# Autodesk Inventor assembly: Assembly1
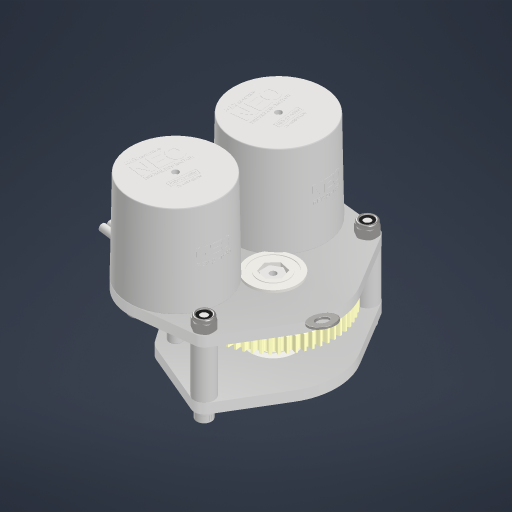
[picture p0: Inventor's stored thumbnail of the model, 512x512]
Saved by Autodesk Inventor 2024.3 (Build 283343000, 343)
## iProperties
Created: 2024-11-01
Part Number: Assembly1
Document SubType Name: Assembly
Designer: kaito
Author: kaito
## Documents named in this file (14)
- C:\Users\kaito\OneDrive\Documents\GitHub\1622-2024-Assignments\Kaito Kubota-Valme\Gearbox 2 v.2\Assembly1.iam
- C:\Users\kaito\OneDrive\Documents\GitHub\1622-2024-Assignments\Kaito Kubota-Valme\Gearbox 2 v.2\Bottom Plate.ipt
- C:\Users\kaito\OneDrive\Documents\GitHub\1622-2024-Assignments\Kaito Kubota-Valme\Gearbox 2 v.2\Part1.ipt
- C:\Users\kaito\OneDrive\Desktop\COTS Library\Motion\Bearings\COTS_WCP-0783_1.125ODHexBearing.ipt
- C:\Users\kaito\OneDrive\Desktop\COTS Library\Motion\Gears\Motor Gears\COTS_217-6334_10T20DPMotorGear.ipt
- C:\Users\kaito\Downloads\REV-21-1650-V1.1\REV-21-1650-V1.1\REV-21-1650-V1.1.ipt
- C:\Users\kaito\OneDrive\Documents\GitHub\1622-2024-Assignments\Kaito Kubota-Valme\Gearbox 2 v.2\Standoff.ipt
- C:\Users\kaito\OneDrive\Documents\GitHub\1622-2024-Assignments\Kaito Kubota-Valme\Gearbox 2 v.2\Hex Shaft.ipt
- C:\Users\kaito\Downloads\WCP-0720 (2)\WCP-0720 (2)\WCP-0720 (2).ipt
- C:\Users\kaito\OneDrive\Desktop\COTS Library\Fasteners\Bolts\Button-Head\10-32\COTS_92949A263_3-8in long Stainless Steel Button Head Screw.ipt
- C:\Users\kaito\OneDrive\Desktop\COTS Library\Fasteners\Washers\COTS_90107A029_316 Stainless Steel Washer.ipt
- C:\Users\kaito\Downloads\91251A550_Black-Oxide Alloy Steel Socket Head Screw\91251A550_Black-Oxide Alloy Steel Socket Head Screw\91251A550_Black-Oxide Alloy Steel Socket Head Screw.ipt
- C:\Users\kaito\OneDrive\Documents\GitHub\1622-2024-Assignments\COTS Library\Fasteners\Nuts\COTS_95615A120_Medium-Strength Steel Nylon-Insert Locknut.ipt
- C:\Users\kaito\OneDrive\Documents\GitHub\1622-2024-Assignments\COTS Library\Fasteners\Washers\COTS_90107A029_316 Stainless Steel Washer.ipt
## Components (28 placed, 12 different names)
1. Bottom Plate:1 — Mate:5, Mate:15, Mate:16, Mate:17, Mate:19, Mate:21, Mate:24, Mate:25, Mate:45, Mate:47, Mate:49
2. Part1:1 — Mate:2, Mate:3, Mate:5, Mate:6, Mate:7, Mate:8, Mate:9, Mate:10, Mate:12, Mate:14, Mate:17, Mate:18, Mate:20, Mate:22, Mate:23, Mate:29, Mate:30, Mate:31, Mate:32, Mate:33, Mate:34, Mate:35, Mate:36, Mate:37, Mate:38, Mate:39, Mate:40, Mate:51, Mate:53, Mate:55
3. COTS_WCP-0783_1.125ODHexBearing:1 — Mate:2, Mate:3, Mate:28
4. COTS_217-6334_10T20DPMotorGear:1 — Mate:13, Mate:14
5. COTS_217-6334_10T20DPMotorGear:2 — Mate:11, Mate:12
6. REV-21-1650-V1.1:1 — Mate:6, Mate:7, Mate:8, Mate:11
7. REV-21-1650-V1.1:2 — Mate:9, Mate:10, Mate:13, Mate:23
8. Standoff:1 — Mate:21, Mate:22, Mate:44
9. Standoff:2 — Mate:15, Mate:16, Mate:18, Mate:48
10. Standoff:3 — Mate:19, Mate:20, Mate:46
11. Hex Shaft:1 — Mate:26, Flush:1, Mate:27, Rotation:1, Mate:42
12. COTS_WCP-0783_1.125ODHexBearing:2 — Mate:24, Mate:25, Mate:26, Flush:1, Mate:41
13. WCP-0720 (2):1 — Mate:27, Mate:28
14. COTS_92949A263_3-8in long Stainless Steel Button Head Screw:1 — Mate:29, Mate:30
15. COTS_92949A263_3-8in long Stainless Steel Button Head Screw:2 — Mate:42, Mate:43
16. COTS_92949A263_3-8in long Stainless Steel Button Head Screw:4 — Mate:31, Mate:32
17. COTS_92949A263_3-8in long Stainless Steel Button Head Screw:5 — Mate:39, Mate:40
18. COTS_92949A263_3-8in long Stainless Steel Button Head Screw:6 — Mate:37, Mate:38
19. COTS_92949A263_3-8in long Stainless Steel Button Head Screw:7 — Mate:35, Mate:36
20. COTS_92949A263_3-8in long Stainless Steel Button Head Screw:8 — Mate:33, Mate:34
21. COTS_90107A029_316 Stainless Steel Washer:1 — Rotation:1, Mate:41, Mate:43
22. 91251A550_Black-Oxide Alloy Steel Socket Head Screw:1 — Mate:44, Mate:45, Mate:54
23. 91251A550_Black-Oxide Alloy Steel Socket Head Screw:2 — Mate:46, Mate:47, Mate:50
24. 91251A550_Black-Oxide Alloy Steel Socket Head Screw:3 — Mate:48, Mate:49, Mate:52
25. COTS_95615A120_Medium-Strength Steel Nylon-Insert Locknut:1 — Mate:50, Mate:51
26. COTS_95615A120_Medium-Strength Steel Nylon-Insert Locknut:2 — Mate:54, Mate:55
27. COTS_95615A120_Medium-Strength Steel Nylon-Insert Locknut:3 — Mate:52, Mate:53
28. COTS_90107A029_316 Stainless Steel Washer:2
## Relationships (55: Mate 53, Flush 1, RelateRotation 1)
- Mate:2: Part1:1 ↔ COTS_WCP-0783_1.125ODHexBearing:1
- Mate:3: Part1:1 ↔ COTS_WCP-0783_1.125ODHexBearing:1
- Mate:5: Bottom Plate:1 ↔ Part1:1
- Mate:6: Part1:1 ↔ REV-21-1650-V1.1:1
- Mate:7: Part1:1 ↔ REV-21-1650-V1.1:1
- Mate:8: Part1:1 ↔ REV-21-1650-V1.1:1
- Mate:9: Part1:1 ↔ REV-21-1650-V1.1:2
- Mate:10: Part1:1 ↔ REV-21-1650-V1.1:2
- Mate:11: COTS_217-6334_10T20DPMotorGear:2 ↔ REV-21-1650-V1.1:1
- Mate:12: Part1:1 ↔ COTS_217-6334_10T20DPMotorGear:2
- Mate:13: COTS_217-6334_10T20DPMotorGear:1 ↔ REV-21-1650-V1.1:2
- Mate:14: Part1:1 ↔ COTS_217-6334_10T20DPMotorGear:1
- Mate:15: Bottom Plate:1 ↔ Standoff:2
- Mate:16: Bottom Plate:1 ↔ Standoff:2
- Mate:17: Bottom Plate:1 ↔ Part1:1
- Mate:18: Part1:1 ↔ Standoff:2
- Mate:19: Bottom Plate:1 ↔ Standoff:3
- Mate:20: Part1:1 ↔ Standoff:3
- Mate:21: Bottom Plate:1 ↔ Standoff:1
- Mate:22: Part1:1 ↔ Standoff:1
- Mate:23: Part1:1 ↔ REV-21-1650-V1.1:2
- Mate:24: Bottom Plate:1 ↔ COTS_WCP-0783_1.125ODHexBearing:2
- Mate:25: Bottom Plate:1 ↔ COTS_WCP-0783_1.125ODHexBearing:2
- Mate:26: Hex Shaft:1 ↔ COTS_WCP-0783_1.125ODHexBearing:2
- Flush:1: Hex Shaft:1 ↔ COTS_WCP-0783_1.125ODHexBearing:2
- Mate:27: Hex Shaft:1 ↔ WCP-0720 (2):1
- Mate:28: COTS_WCP-0783_1.125ODHexBearing:1 ↔ WCP-0720 (2):1
- Mate:29: Part1:1 ↔ COTS_92949A263_3-8in long Stainless Steel Button Head Screw:1
- Mate:30: Part1:1 ↔ COTS_92949A263_3-8in long Stainless Steel Button Head Screw:1
- Mate:31: Part1:1 ↔ COTS_92949A263_3-8in long Stainless Steel Button Head Screw:4
- Mate:32: Part1:1 ↔ COTS_92949A263_3-8in long Stainless Steel Button Head Screw:4
- Mate:33: Part1:1 ↔ COTS_92949A263_3-8in long Stainless Steel Button Head Screw:8
- Mate:34: Part1:1 ↔ COTS_92949A263_3-8in long Stainless Steel Button Head Screw:8
- Mate:35: Part1:1 ↔ COTS_92949A263_3-8in long Stainless Steel Button Head Screw:7
- Mate:36: Part1:1 ↔ COTS_92949A263_3-8in long Stainless Steel Button Head Screw:7
- Mate:37: Part1:1 ↔ COTS_92949A263_3-8in long Stainless Steel Button Head Screw:6
- Mate:38: Part1:1 ↔ COTS_92949A263_3-8in long Stainless Steel Button Head Screw:6
- Mate:39: Part1:1 ↔ COTS_92949A263_3-8in long Stainless Steel Button Head Screw:5
- Mate:40: Part1:1 ↔ COTS_92949A263_3-8in long Stainless Steel Button Head Screw:5
- Rotation:1 [RelateRotation] (1.767 ul): Hex Shaft:1 ↔ COTS_90107A029_316 Stainless Steel Washer:1
- Mate:41: COTS_WCP-0783_1.125ODHexBearing:2 ↔ COTS_90107A029_316 Stainless Steel Washer:1
- Mate:42: Hex Shaft:1 ↔ COTS_92949A263_3-8in long Stainless Steel Button Head Screw:2
- Mate:43: COTS_92949A263_3-8in long Stainless Steel Button Head Screw:2 ↔ COTS_90107A029_316 Stainless Steel Washer:1
- Mate:44: Standoff:1 ↔ 91251A550_Black-Oxide Alloy Steel Socket Head Screw:1
- Mate:45: Bottom Plate:1 ↔ 91251A550_Black-Oxide Alloy Steel Socket Head Screw:1
- Mate:46: Standoff:3 ↔ 91251A550_Black-Oxide Alloy Steel Socket Head Screw:2
- Mate:47: Bottom Plate:1 ↔ 91251A550_Black-Oxide Alloy Steel Socket Head Screw:2
- Mate:48: Standoff:2 ↔ 91251A550_Black-Oxide Alloy Steel Socket Head Screw:3
- Mate:49: Bottom Plate:1 ↔ 91251A550_Black-Oxide Alloy Steel Socket Head Screw:3
- Mate:50: 91251A550_Black-Oxide Alloy Steel Socket Head Screw:2 ↔ COTS_95615A120_Medium-Strength Steel Nylon-Insert Locknut:1
- Mate:51: Part1:1 ↔ COTS_95615A120_Medium-Strength Steel Nylon-Insert Locknut:1
- Mate:52: 91251A550_Black-Oxide Alloy Steel Socket Head Screw:3 ↔ COTS_95615A120_Medium-Strength Steel Nylon-Insert Locknut:3
- Mate:53: Part1:1 ↔ COTS_95615A120_Medium-Strength Steel Nylon-Insert Locknut:3
- Mate:54: 91251A550_Black-Oxide Alloy Steel Socket Head Screw:1 ↔ COTS_95615A120_Medium-Strength Steel Nylon-Insert Locknut:2
- Mate:55: Part1:1 ↔ COTS_95615A120_Medium-Strength Steel Nylon-Insert Locknut:2
